# Autodesk Inventor assembly: Assembly1_TT
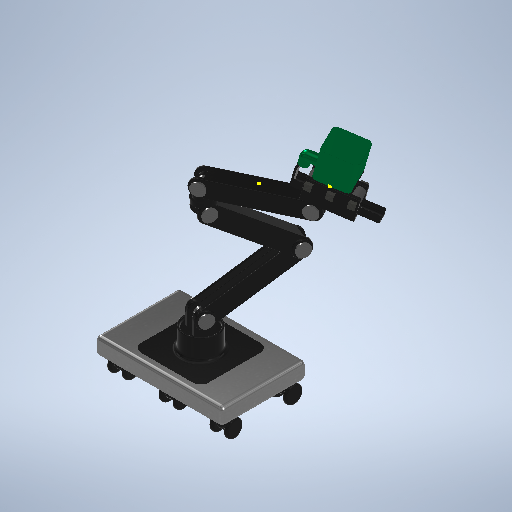
[picture p0: Inventor's stored thumbnail of the model, 512x512]
Saved by Autodesk Inventor 2027.1 (Build 311270010, 270A)
## iProperties
Created: 2026-08-27
Part Number: Assembly1_TT
Document SubType Name: Assembly
Designer: RIDDHIMAN
Author: RIDDHIMAN
## Documents named in this file (16)
- D:\ZINE ROUND 2\MULTI-DOF_TT_ROBOT.iam
- D:\ZINE ROUND 2\HAND_BASE2.ipt
- D:\ZINE ROUND 2\ARM1.ipt
- D:\ZINE ROUND 2\ARM2.ipt
- D:\ZINE ROUND 2\HAND_BASE1.ipt
- D:\ZINE ROUND 2\joint1.ipt
- D:\ZINE ROUND 2\joint2.ipt
- D:\ZINE ROUND 2\JOINT_BASE2.ipt
- D:\ZINE ROUND 2\JOINT_BASE1.ipt
- D:\ZINE ROUND 2\SHOOTING_GUN.ipt
- D:\ZINE ROUND 2\ROLLER_SHAFT.ipt
- D:\ZINE ROUND 2\ROLLER.ipt
- D:\ZINE ROUND 2\STORAGE_BASKET.ipt
- D:\ZINE ROUND 2\WHEEL_BASE.ipt
- D:\ZINE ROUND 2\WHEEL_JOINT.ipt
- D:\ZINE ROUND 2\WHEEL.ipt
## Components (33 placed, 15 different names)
1. HAND_BASE2:1 — Rotational:3, Rigid:16
2. ARM1:1 — Rotational:1, Rotational:2, Rigid:2
3. ARM2:1 — Rotational:2, Rigid:1, Rigid:3, Rotational:4
4. HAND_BASE1:1 — Rotational:1, Rotational:3
5. joint1:1 — Rigid:1
6. joint1:2 — Rigid:2
7. joint2:1 — Rigid:3
8. JOINT_BASE2:1 — Rotational:5, Rotational:6
9. ARM2:2 — Rotational:6, Rigid:4, Rotational:7
10. JOINT_BASE1:1 — Rotational:4, Rotational:5
11. joint2:2 — Rigid:4
12. SHOOTING_GUN:1 — Rotational:7, Rigid:5, Rigid:6, Rigid:7, Rigid:8, Rigid:9
13. joint2:3 — Rigid:5
14. ROLLER_SHAFT:1 — Rotational:8, Rigid:6
15. ROLLER:1 — Rotational:8
16. ROLLER_SHAFT:2 — Rigid:7
17. ROLLER:2
18. ROLLER_SHAFT:3 — Rigid:8
19. ROLLER:3
20. STORAGE_BASKET:1 — Rigid:9
21. WHEEL_BASE:1 — Rotational:11, Rotational:12, Rotational:13, Rotational:14, Rotational:15, Rotational:16, Rigid:16
22. WHEEL_JOINT:1 — Rigid:10, Rotational:11
23. WHEEL:1 — Rigid:10
24. WHEEL_JOINT:2 — Rotational:13
25. WHEEL:2
26. WHEEL_JOINT:3 — Rotational:14
27. WHEEL:3
28. WHEEL_JOINT:4 — Rotational:12
29. WHEEL:4
30. WHEEL_JOINT:5 — Rotational:16
31. WHEEL:5
32. WHEEL_JOINT:6 — Rotational:15
33. WHEEL:6
## Relationships (32: RevoluteJoint 16, WeldJoint 16)
- Rotational:1 [RevoluteJoint]: ARM1:1 ↔ HAND_BASE1:1
- Rotational:2 [RevoluteJoint]: ARM1:1 ↔ ARM2:1
- Rotational:3 [RevoluteJoint]: HAND_BASE2:1 ↔ HAND_BASE1:1
- Rigid:1 [WeldJoint]: ARM2:1 ↔ joint1:1
- Rigid:2 [WeldJoint]: ARM1:1 ↔ joint1:2
- Rigid:3 [WeldJoint]: ARM2:1 ↔ joint2:1
- Rotational:4 [RevoluteJoint]: ARM2:1 ↔ JOINT_BASE1:1
- Rotational:5 [RevoluteJoint]: JOINT_BASE2:1 ↔ JOINT_BASE1:1
- Rotational:6 [RevoluteJoint]: JOINT_BASE2:1 ↔ ARM2:2
- Rigid:4 [WeldJoint]: ARM2:2 ↔ joint2:2
- Rotational:7 [RevoluteJoint]: ARM2:2 ↔ SHOOTING_GUN:1
- Rigid:5 [WeldJoint]: SHOOTING_GUN:1 ↔ joint2:3
- Rotational:8 [RevoluteJoint]: ROLLER_SHAFT:1 ↔ ROLLER:1
- Rigid:6 [WeldJoint]: SHOOTING_GUN:1 ↔ ROLLER_SHAFT:1
- [RevoluteJoint]: ROLLER_SHAFT:2 ↔ ROLLER:2
- Rigid:7 [WeldJoint]: SHOOTING_GUN:1 ↔ ROLLER_SHAFT:2
- [RevoluteJoint]: ROLLER_SHAFT:3 ↔ ROLLER:3
- Rigid:8 [WeldJoint]: SHOOTING_GUN:1 ↔ ROLLER_SHAFT:3
- Rigid:9 [WeldJoint]: SHOOTING_GUN:1 ↔ STORAGE_BASKET:1
- Rigid:10 [WeldJoint]: WHEEL_JOINT:1 ↔ WHEEL:1
- [WeldJoint]: WHEEL_JOINT:2 ↔ WHEEL:2
- [WeldJoint]: WHEEL_JOINT:3 ↔ WHEEL:3
- [WeldJoint]: WHEEL_JOINT:4 ↔ WHEEL:4
- [WeldJoint]: WHEEL_JOINT:5 ↔ WHEEL:5
- [WeldJoint]: WHEEL_JOINT:6 ↔ WHEEL:6
- Rotational:11 [RevoluteJoint]: WHEEL_BASE:1 ↔ WHEEL_JOINT:1
- Rotational:12 [RevoluteJoint]: WHEEL_BASE:1 ↔ WHEEL_JOINT:4
- Rotational:13 [RevoluteJoint]: WHEEL_BASE:1 ↔ WHEEL_JOINT:2
- Rotational:14 [RevoluteJoint]: WHEEL_BASE:1 ↔ WHEEL_JOINT:3
- Rotational:15 [RevoluteJoint]: WHEEL_BASE:1 ↔ WHEEL_JOINT:6
- Rotational:16 [RevoluteJoint]: WHEEL_BASE:1 ↔ WHEEL_JOINT:5
- Rigid:16 [WeldJoint]: HAND_BASE2:1 ↔ WHEEL_BASE:1
## Named parameters: d45_d40 = 0 mm, d46_d41 = -167.424614 deg, d48_d40 = 0 mm, d49_d41 = -10.224258 deg, d53_d52 = 0 mm, d54_d52 = 0 mm, d55_d52 = 0 mm, d56_d52 = 0 mm, d57_d52 = 0 mm
